# Autodesk Inventor assembly: vwheel
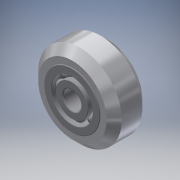
[picture p0: Inventor's stored thumbnail of the model, 180x180]
Saved by Autodesk Inventor 2016 (Build 200138000, 138)
## iProperties
Created: 2016-03-19
Part Number: vwheel
Document SubType Name: Assembly
Designer: Solomon
Author: Solomon
## Documents named in this file (3)
- C:\Users\Solomon\Documents\Inventor\SLA MK I\vwheel.iam
- C:\Users\Solomon\Documents\Inventor\SLA MK I\V Slot Part Files\Pulleys Wheels Bearings\Solid V Wheel.ipt
- C:\Users\Solomon\Documents\Inventor\SLA MK I\5mm-bearing\5mm Bearing SKF 625 (RS 286-7811).ipt
## Components (3 placed, 2 different names)
1. Solid V Wheel:1 — Angle:1, Insert:1, Tangent:1, Flush:1
2. 5mm Bearing SKF 625 (RS 286-7811):1 — Angle:1, Insert:1, Angle:2
3. 5mm Bearing SKF 625 (RS 286-7811):2 — Angle:2, Tangent:1, Flush:1
## Relationships (5: Angle 2, Insert 1, Tangent 1, Flush 1)
- Angle:1 (0 deg): Solid V Wheel:1 ↔ 5mm Bearing SKF 625 (RS 286-7811):1
- Insert:1: Solid V Wheel:1 ↔ 5mm Bearing SKF 625 (RS 286-7811):1
- Angle:2 (0 deg): 5mm Bearing SKF 625 (RS 286-7811):1 ↔ 5mm Bearing SKF 625 (RS 286-7811):2
- Tangent:1: Solid V Wheel:1 ↔ 5mm Bearing SKF 625 (RS 286-7811):2
- Flush:1: Solid V Wheel:1 ↔ 5mm Bearing SKF 625 (RS 286-7811):2
